# Autodesk Inventor assembly: Final2
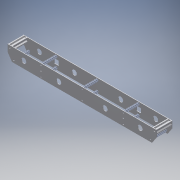
[picture p0: Inventor's stored thumbnail of the model, 180x180]
Saved by Autodesk Inventor 2016 (Build 200138000, 138)
## iProperties
Created: 2017-01-21
Part Number: Final2
Document SubType Name: Assembly
Designer: hamblettk
Author: hamblettk
## Documents named in this file (5)
- E:\1073CAD\Robot2017\DriveTrain\Final2.iam
- E:\1073CAD\Robot2017\DriveTrain\OutsidePlate2.ipt
- E:\1073CAD\Robot2017\DriveTrain\Individual Parts\3.625Churro.ipt
- E:\1073CAD\Robot2017\DriveTrain\Individual Parts\Mock 8020 3.375in.ipt
- E:\1073CAD\Robot2017\DriveTrain\InsidePlate2.ipt
## Components (12 placed, 4 different names)
1. OutsidePlate2:1 — Mate:1, Mate:2, Mate:3, Mate:4, Mate:5, Mate:6, Mate:7, Mate:8, Mate:9, Mate:10, Flush:1, Flush:2
2. 3.625Churro:1 — Mate:1
3. 3.625Churro:2 — Mate:8
4. 3.625Churro:3 — Mate:7
5. 3.625Churro:4 — Mate:6
6. 3.625Churro:5 — Mate:4
7. 3.625Churro:6 — Mate:5
8. 3.625Churro:7 — Mate:2
9. 3.625Churro:8 — Mate:3
10. Mock 8020 3.375in:1 — Mate:9, Mate:11
11. Mock 8020 3.375in:2 — Mate:10
12. InsidePlate2:1 — Mate:11, Flush:1, Flush:2
## Relationships (13: Mate 11, Flush 2)
- Mate:1: OutsidePlate2:1 ↔ 3.625Churro:1
- Mate:2: OutsidePlate2:1 ↔ 3.625Churro:7
- Mate:3: OutsidePlate2:1 ↔ 3.625Churro:8
- Mate:4: OutsidePlate2:1 ↔ 3.625Churro:5
- Mate:5: OutsidePlate2:1 ↔ 3.625Churro:6
- Mate:6: OutsidePlate2:1 ↔ 3.625Churro:4
- Mate:7: OutsidePlate2:1 ↔ 3.625Churro:3
- Mate:8: OutsidePlate2:1 ↔ 3.625Churro:2
- Mate:9: OutsidePlate2:1 ↔ Mock 8020 3.375in:1
- Mate:10: OutsidePlate2:1 ↔ Mock 8020 3.375in:2
- Mate:11: Mock 8020 3.375in:1 ↔ InsidePlate2:1
- Flush:1: OutsidePlate2:1 ↔ InsidePlate2:1
- Flush:2: OutsidePlate2:1 ↔ InsidePlate2:1
